# Autodesk Inventor assembly: string holder
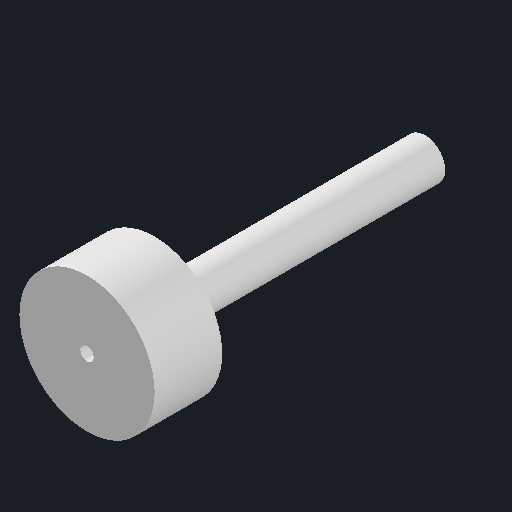
[picture p0: Inventor's stored thumbnail of the model, 512x512]
Saved by Autodesk Inventor 2026 (Build 300175050, 175E)
## iProperties
Created: 2025-10-28
Part Number: string holder
Document SubType Name: Assembly
Designer: sachd
Author: sachd
## Documents named in this file (3)
- C:\Users\exp-213\Desktop\Final Deliverable CA\string holder.iam
- C:\Users\exp-213\Desktop\Final Deliverable CA\string holder base.ipt
- C:\Users\exp-213\Desktop\Final Deliverable CA\string holder head.ipt
## Components (2 placed, 2 different names)
1. string holder base:1 — Insert:1, Flush:1
2. string holder head:1 — Insert:1, Flush:1
## Relationships (2: Insert 1, Flush 1)
- Insert:1: string holder base:1 ↔ string holder head:1
- Flush:1: string holder base:1 ↔ string holder head:1
